# Autodesk Inventor assembly: HDMI-Female-PanelMount
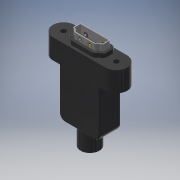
[picture p0: Inventor's stored thumbnail of the model, 180x180]
Saved by Autodesk Inventor 2017 (Build 210142000, 142)
## iProperties
Created: 2020-10-05
Part Number: HDMI-Female-PanelMount
Document SubType Name: Assembly
Designer: Joe Ferner
Author: Joe Ferner
## Documents named in this file (3)
- C:\dev\raspberry-pi-ir-hat\models3d\HDMI-Female-PanelMount\HDMI-Female-PanelMount.iam
- C:\dev\raspberry-pi-ir-hat\models3d\HDMI-Female-PanelMount\hdmi-port.ipt
- C:\dev\raspberry-pi-ir-hat\models3d\HDMI-Female-PanelMount\hdmi-panel-mount.ipt
## Components (2 placed, 2 different names)
1. hdmi-port:1 — Flush:1, Mate:1, Mate:2
2. hdmi-panel-mount:1 — Flush:1, Mate:1, Mate:2
## Relationships (3: Mate 2, Flush 1)
- Flush:1 (5 mm): hdmi-port:1 ↔ hdmi-panel-mount:1
- Mate:1: hdmi-port:1 ↔ hdmi-panel-mount:1
- Mate:2: hdmi-port:1 ↔ hdmi-panel-mount:1
